# Autodesk Inventor assembly: Property
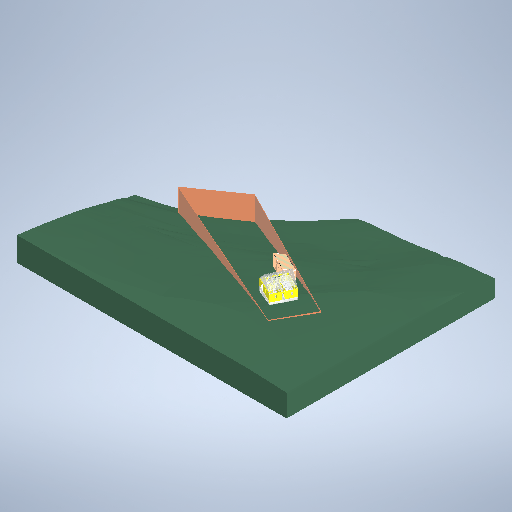
[picture p0: Inventor's stored thumbnail of the model, 512x512]
Saved by Autodesk Inventor 2025.1 (Build 291241020, 241B)
## iProperties
Created: 2023-06-05
Part Number: Property
Document SubType Name: Assembly
Designer: Tom
Author: Tom
## Documents named in this file (5)
- C:\Users\Tom\Documents\Inventor\Mobility\Property.iam
- C:\Users\Tom\Documents\Inventor\Mobility\Land.ipt
- C:\Users\Tom\Documents\Inventor\Mobility\Fence.ipt
- C:\Users\Tom\Documents\Inventor\Mobility\Finished_House.iam
- C:\Users\Tom\Documents\Inventor\Mobility\Additional_Building\Additional_Building.iam
## Components (4 placed, 4 different names)
1. Land:1 — Flush:1, Mate:1, Mate:2
2. Fence:1
3. Finished_House:1 [sub-assembly] — Flush:1, Mate:1, Mate:2, Mate:3, Mate:4, Mate:5
4. Additional_Building:1 [sub-assembly] — Mate:3, Mate:4, Mate:5
## Relationships (6: Mate 5, Flush 1)
- Flush:1 (6248.4 mm): Land:1 ↔ Finished_House:1
- Mate:1 (12.7 mm): Land:1 ↔ Finished_House:1
- Mate:2 (228.6 mm): Land:1 ↔ Finished_House:1
- Mate:3 (3189.2875 mm): Finished_House:1 ↔ Additional_Building:1
- Mate:4: Finished_House:1 ↔ Additional_Building:1
- Mate:5: Finished_House:1 ↔ Additional_Building:1
